# Autodesk Inventor assembly: 040102 DR-18-H8_CPY
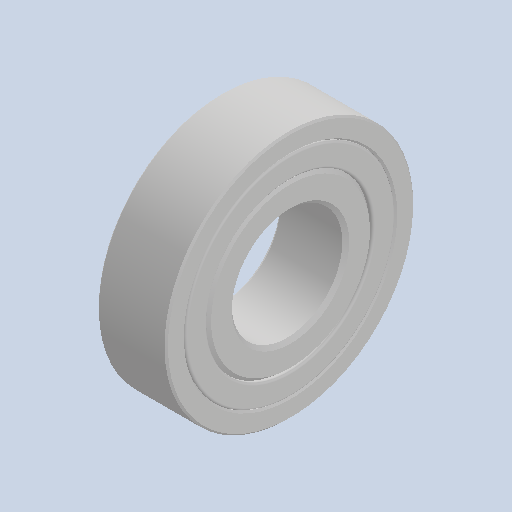
[picture p0: Inventor's stored thumbnail of the model, 512x512]
Saved by Autodesk Inventor 2024 (Build 280153000, 153)
## iProperties
Category: PARTsolutions
Created: 2023-06-20
Part Number: 040102 DR-18-H8_CPY
Catalog Web Link: www.cadenas.de
Description: DR-H-
Document SubType Name: Assembly
Designer: zegi
Mass: 78300 g
Surface Area: 16.8912 cm^2
Volume: 0.803937 cm^3
Density: 97395.6 g/cm^3
Title: 040102 DR-18-H8
Author: Cadenas PARTsolutions
PSOL_IDENT_0: {$CADENAS_DATA/23d-libs/tok_bearing/d_series_bearings/dr_h_asmtab.prj},175 {VTYP=3D},{STYP=ASSTAB},{
PSOL_IDENT_1: NB=040102 DR-18-H8},{LINA=040102 DR-18-H8},{NN=DR-H},{DATE=16.12.2020 00:38:04},{GEOMDATE=19.02.2013
PSOL_IDENT_2: },{VERSION=},{LINEID=1710},{WBVAR=},{WBNUMERIC=}  {NB=040102 DR-18-H8},{LINA=040102 DR-18-H8},{KT=DU
PSOL_IDENT_3: MMY},{IDNR=},{CODE=040102},{PN=DR-18-H8},{D=18},{SD=8.0},{W=5.0},{W1=-},{W1X=0.000},{W2=-},{W2X=0.00
PSOL_IDENT_4: 0},{LOAD=49 (5)},{TYPE=11},{QTY=3.000},{GW=8.7},{BD=3.2},{OP=42.704},{N=6},{R=6.8},{GP=1.4},{PPATH=d
PSOL_IDENT_5: r_h/dr_h_asmtpl.prj}
NB: 040102 DR-18-H8
NN: DR-H
NBSYN: $CODE. $PN.
LINA: 040102 DR-18-H8
CATALOG: TOK, Inc
CODE: 040102
PN: DR-18-H8
D: 18
SD: 8
W: 5
W1: -
W2: -
LOAD: 49 (5)
TYPE: 11
QTY: 3.000
GW: 8.7
ARTICLENO: 040102 DR-18-H8
BOMINFO: 040102 DR-18-H8
CREATOR: CADENAS GmbH
## Documents named in this file (5)
- C:\Users\zegi\OneDrive - Kyushu University\KURT\2023キャチロボ\cad\000_parts_zegi\bearing\8\DR-18-H8\AIS2023\040102 DR-18-H8_CPY.iam
- C:\Users\zegi\OneDrive - Kyushu University\KURT\2023キャチロボ\cad\000_parts_zegi\bearing\8\DR-18-H8\AIS2023\040102DR-18-H8_ir_CPY.ipt
- C:\Users\zegi\OneDrive - Kyushu University\KURT\2023キャチロボ\cad\000_parts_zegi\bearing\8\DR-18-H8\AIS2023\040102DR-18-H8_or_CPY.ipt
- C:\Users\zegi\OneDrive - Kyushu University\KURT\2023キャチロボ\cad\000_parts_zegi\bearing\8\DR-18-H8\AIS2023\040102DR-18-H8_cage_CPY.ipt
- C:\Users\zegi\OneDrive - Kyushu University\KURT\2023キャチロボ\cad\000_parts_zegi\bearing\8\DR-18-H8\AIS2023\040102DR-18-H8_ball_CPY.ipt
## Components (9 placed, 4 different names)
1. 040102DR-18-H8_ir_CPY:1 — IR_OR_Z@1 <-> OR_IR_Z@2, IR_OR_XY@1 <-> OR_IR_XY@2
2. 040102DR-18-H8_or_CPY:1 — IR_OR_Z@1 <-> OR_IR_Z@2, IR_OR_XY@1 <-> OR_IR_XY@2, OR_IR_Z@2 <-> Cage_OR_Z@3, OR_IR_XY@2 <-> Cage_OR_XY@3, OR_ball_1_Z@2 <-> Ball_OR_Z@4, OR_ball_1_XY@2 <-> Ball_OR_XY@4, OR_ball_2_Z@2 <-> Ball_OR_Z@5, OR_ball_2_XY@2 <-> Ball_OR_XY@5, OR_ball_3_Z@2 <-> Ball_OR_Z@6, OR_ball_3_XY@2 <-> Ball_OR_XY@6, OR_ball_4_Z@2 <-> Ball_OR_Z@7, OR_ball_4_XY@2 <-> Ball_OR_XY@7, OR_ball_5_Z@2 <-> Ball_OR_Z@8, OR_ball_5_XY@2 <-> Ball_OR_XY@8, OR_ball_6_Z@2 <-> Ball_OR_Z@9, OR_ball_6_XY@2 <-> Ball_OR_XY@9, OR_ball_1_YZ@2 <-> Ball_OR_YZ@4, OR_ball_2_YZ@2 <-> Ball_OR_YZ@5, OR_ball_3_YZ@2 <-> Ball_OR_YZ@6, OR_ball_4_YZ@2 <-> Ball_OR_YZ@7, OR_ball_5_YZ@2 <-> Ball_OR_YZ@8, OR_ball_6_YZ@2 <-> Ball_OR_YZ@9
3. 040102DR-18-H8_cage_CPY:1 — OR_IR_Z@2 <-> Cage_OR_Z@3, OR_IR_XY@2 <-> Cage_OR_XY@3
4. 040102DR-18-H8_ball_CPY:1 — OR_ball_1_Z@2 <-> Ball_OR_Z@4, OR_ball_1_XY@2 <-> Ball_OR_XY@4, OR_ball_1_YZ@2 <-> Ball_OR_YZ@4
5. 040102DR-18-H8_ball_CPY:2 — OR_ball_2_Z@2 <-> Ball_OR_Z@5, OR_ball_2_XY@2 <-> Ball_OR_XY@5, OR_ball_2_YZ@2 <-> Ball_OR_YZ@5
6. 040102DR-18-H8_ball_CPY:3 — OR_ball_3_Z@2 <-> Ball_OR_Z@6, OR_ball_3_XY@2 <-> Ball_OR_XY@6, OR_ball_3_YZ@2 <-> Ball_OR_YZ@6
7. 040102DR-18-H8_ball_CPY:4 — OR_ball_4_Z@2 <-> Ball_OR_Z@7, OR_ball_4_XY@2 <-> Ball_OR_XY@7, OR_ball_4_YZ@2 <-> Ball_OR_YZ@7
8. 040102DR-18-H8_ball_CPY:5 — OR_ball_5_Z@2 <-> Ball_OR_Z@8, OR_ball_5_XY@2 <-> Ball_OR_XY@8, OR_ball_5_YZ@2 <-> Ball_OR_YZ@8
9. 040102DR-18-H8_ball_CPY:6 — OR_ball_6_Z@2 <-> Ball_OR_Z@9, OR_ball_6_XY@2 <-> Ball_OR_XY@9, OR_ball_6_YZ@2 <-> Ball_OR_YZ@9
## Relationships (22: Mate 14, Angle 6, Flush 2)
- IR_OR_Z@1 <-> OR_IR_Z@2 [Mate]: 040102DR-18-H8_ir_CPY:1 ↔ 040102DR-18-H8_or_CPY:1
- IR_OR_XY@1 <-> OR_IR_XY@2 [Flush]: 040102DR-18-H8_ir_CPY:1 ↔ 040102DR-18-H8_or_CPY:1
- OR_IR_Z@2 <-> Cage_OR_Z@3 [Mate]: 040102DR-18-H8_or_CPY:1 ↔ 040102DR-18-H8_cage_CPY:1
- OR_IR_XY@2 <-> Cage_OR_XY@3 [Flush]: 040102DR-18-H8_or_CPY:1 ↔ 040102DR-18-H8_cage_CPY:1
- OR_ball_1_Z@2 <-> Ball_OR_Z@4 [Mate]: 040102DR-18-H8_or_CPY:1 ↔ 040102DR-18-H8_ball_CPY:1
- OR_ball_1_XY@2 <-> Ball_OR_XY@4 [Mate]: 040102DR-18-H8_or_CPY:1 ↔ 040102DR-18-H8_ball_CPY:1
- OR_ball_2_Z@2 <-> Ball_OR_Z@5 [Mate]: 040102DR-18-H8_or_CPY:1 ↔ 040102DR-18-H8_ball_CPY:2
- OR_ball_2_XY@2 <-> Ball_OR_XY@5 [Mate]: 040102DR-18-H8_or_CPY:1 ↔ 040102DR-18-H8_ball_CPY:2
- OR_ball_3_Z@2 <-> Ball_OR_Z@6 [Mate]: 040102DR-18-H8_or_CPY:1 ↔ 040102DR-18-H8_ball_CPY:3
- OR_ball_3_XY@2 <-> Ball_OR_XY@6 [Mate]: 040102DR-18-H8_or_CPY:1 ↔ 040102DR-18-H8_ball_CPY:3
- OR_ball_4_Z@2 <-> Ball_OR_Z@7 [Mate]: 040102DR-18-H8_or_CPY:1 ↔ 040102DR-18-H8_ball_CPY:4
- OR_ball_4_XY@2 <-> Ball_OR_XY@7 [Mate]: 040102DR-18-H8_or_CPY:1 ↔ 040102DR-18-H8_ball_CPY:4
- OR_ball_5_Z@2 <-> Ball_OR_Z@8 [Mate]: 040102DR-18-H8_or_CPY:1 ↔ 040102DR-18-H8_ball_CPY:5
- OR_ball_5_XY@2 <-> Ball_OR_XY@8 [Mate]: 040102DR-18-H8_or_CPY:1 ↔ 040102DR-18-H8_ball_CPY:5
- OR_ball_6_Z@2 <-> Ball_OR_Z@9 [Mate]: 040102DR-18-H8_or_CPY:1 ↔ 040102DR-18-H8_ball_CPY:6
- OR_ball_6_XY@2 <-> Ball_OR_XY@9 [Mate]: 040102DR-18-H8_or_CPY:1 ↔ 040102DR-18-H8_ball_CPY:6
- OR_ball_1_YZ@2 <-> Ball_OR_YZ@4 [Angle] (0 deg): 040102DR-18-H8_or_CPY:1 ↔ 040102DR-18-H8_ball_CPY:1
- OR_ball_2_YZ@2 <-> Ball_OR_YZ@5 [Angle] (0 deg): 040102DR-18-H8_or_CPY:1 ↔ 040102DR-18-H8_ball_CPY:2
- OR_ball_3_YZ@2 <-> Ball_OR_YZ@6 [Angle] (0 deg): 040102DR-18-H8_or_CPY:1 ↔ 040102DR-18-H8_ball_CPY:3
- OR_ball_4_YZ@2 <-> Ball_OR_YZ@7 [Angle] (0 deg): 040102DR-18-H8_or_CPY:1 ↔ 040102DR-18-H8_ball_CPY:4
- OR_ball_5_YZ@2 <-> Ball_OR_YZ@8 [Angle] (0 deg): 040102DR-18-H8_or_CPY:1 ↔ 040102DR-18-H8_ball_CPY:5
- OR_ball_6_YZ@2 <-> Ball_OR_YZ@9 [Angle] (0 deg): 040102DR-18-H8_or_CPY:1 ↔ 040102DR-18-H8_ball_CPY:6
